# Autodesk Inventor assembly: banner
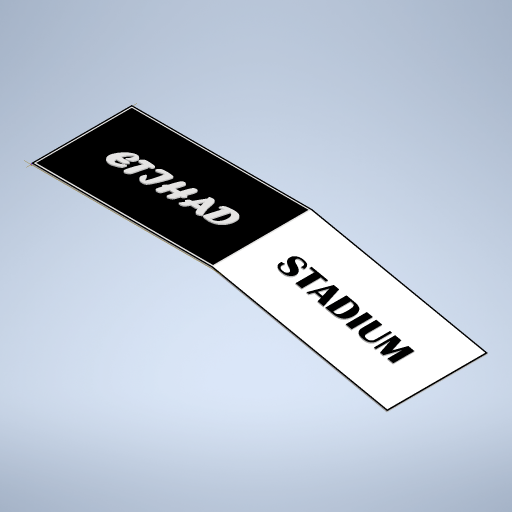
[picture p0: Inventor's stored thumbnail of the model, 512x512]
Saved by Autodesk Inventor 2024.1 (Build 281209000, 209)
## iProperties
Created: 2023-11-18
Part Number: banner
Document SubType Name: Assembly
Designer: ASUS
Author: ASUS
## Documents named in this file (3)
- C:\EAH\HK1_Nam4\IE402-3C\Etihad\EtihadStadium-3D\model\banner\banner.iam
- C:\EAH\HK1_Nam4\IE402-3C\Etihad\EtihadStadium-3D\model\banner\banner1.ipt
- C:\EAH\HK1_Nam4\IE402-3C\Etihad\EtihadStadium-3D\model\banner\banner2.ipt
## Components (2 placed, 2 different names)
1. banner1:1 — Mate:1, Mate:2, Mate:3, Mate:4
2. banner2:1 — Mate:1
## Relationships (4: Mate 4)
- Mate:1: banner1:1 ↔ banner2:1
- Mate:2: banner1:1
- Mate:3: banner1:1
- Mate:4: banner1:1
